# Autodesk Inventor assembly: Digit
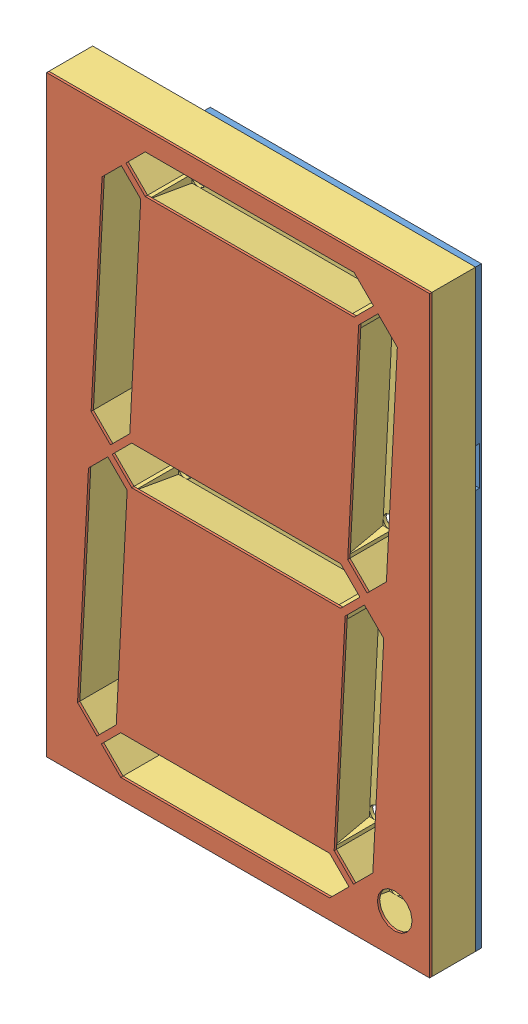
[picture p0: shaded view drawn from the part files that the assembly names]
Saved by Autodesk Inventor 2016 SP2 (Build 200236200, 236)
## iProperties
Created: 2018-10-04
Part Number: Digit
Material: Generisch
Document SubType Name: Assembly
Designer: Nils
Author: Nils
## Documents named in this file (4)
- C:\Users\Nils\Documents\Projects\Big Stopwatch\Big-Stopwatch\Models\Counter\Digit.iam
- C:\Users\Nils\Documents\Projects\Big Stopwatch\Big-Stopwatch\Models\Counter\Backplate_V2.ipt
- C:\Users\Nils\Documents\Projects\Big Stopwatch\Big-Stopwatch\Models\Counter\Cover_V2.ipt
- C:\Users\Nils\Documents\Projects\Big Stopwatch\Big-Stopwatch\Models\Counter\Segment_V4.ipt
## Components (3 placed, 3 different names)
1. Backplate_V2:1 — Fluchtend:3, Fluchtend:4, Passend:2
2. Cover_V2:1 — Fluchtend:1, Fluchtend:2, Passend:1
3. Segment_V4:1 — Fluchtend:1, Fluchtend:2, Fluchtend:3, Fluchtend:4, Passend:1, Passend:2
## Relationships (6: Flush 4, Mate 2)
- Fluchtend:1 [Flush]: Cover_V2:1 ↔ Segment_V4:1
- Fluchtend:2 [Flush]: Cover_V2:1 ↔ Segment_V4:1
- Fluchtend:3 [Flush]: Backplate_V2:1 ↔ Segment_V4:1
- Fluchtend:4 [Flush]: Backplate_V2:1 ↔ Segment_V4:1
- Passend:1 [Mate]: Cover_V2:1 ↔ Segment_V4:1
- Passend:2 [Mate]: Backplate_V2:1 ↔ Segment_V4:1
